# Autodesk Inventor assembly: _Fishing Rod Assembly
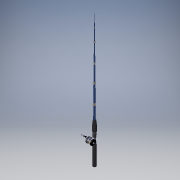
[picture p0: Inventor's stored thumbnail of the model, 180x180]
Saved by Autodesk Inventor 2019 (Build 230136000, 136)
## iProperties
Company: Autodesk
Created: 2017-06-16
Part Number: _Fishing Rod Assembly
Document SubType Name: Assembly
Designer: Autodesk
Mass: 363.885 g
Surface Area: 2982.93 cm^2
Volume: 868.927 cm^3
Density: 0.418775 g/cm^3
Author: Inventor
## Documents named in this file (3)
- C:\TEMP\Fishing Rod\Workspaces\_Fishing Rod Assembly.iam
- C:\TEMP\Fishing Rod\Workspaces\Rod Assembly.iam
- C:\TEMP\Fishing Rod\Workspaces\_Fishing Reel Assembly.iam
## Components (2 placed, 2 different names)
1. Rod Assembly:1 [sub-assembly] — Mate:1, Mate:2
2. _Fishing Reel Assembly:1 [sub-assembly] — Mate:1, Angle:1, Mate:2, Angle:2
## Relationships (4: Mate 2, Angle 2)
- Mate:1: Rod Assembly:1 ↔ _Fishing Reel Assembly:1
- Angle:1 (180 deg): _Fishing Reel Assembly:1
- Mate:2 (14 mm): Rod Assembly:1 ↔ _Fishing Reel Assembly:1
- Angle:2: _Fishing Reel Assembly:1
